# Autodesk Inventor assembly: xy forearm
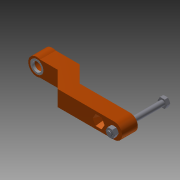
[picture p0: Inventor's stored thumbnail of the model, 180x180]
Saved by Autodesk Inventor 2014 (Build 180170000, 170)
## iProperties
Created: 2013-10-15
Part Number: xy forearm
Document SubType Name: Assembly
Designer: employee
Author: employee
## Documents named in this file (6)
- \\GRISTLE\speco\GitHub\ConceptFORGE\Wally\xy forearm.iam
- \\GRISTLE\speco\GitHub\ConceptFORGE\Wally\xy forearm.ipt
- \\GRISTLE\speco\GitHub\ConceptFORGE\Wally\M3x16.ipt
- \\GRISTLE\speco\GitHub\ConceptFORGE\Wally\6702.ipt
- \\GRISTLE\speco\GitHub\ConceptFORGE\Wally\M8 nut.ipt
- \\GRISTLE\speco\GitHub\ConceptFORGE\Wally\M8x85.ipt
## Components (6 placed, 5 different names)
1. xy forearm:1 — Insert:1, Insert:2, Insert:3, Insert:4, Insert:5
2. Forged Socket Head Cap Screw - Metric M3x0.5 x 16:1 — Insert:1
3. 6702:1 — Insert:2
4. 6702:2 — Insert:3
5. Hex Nut Metric M8 x 1.25:1 — Insert:4
6. M8x85 — Insert:5
## Relationships (5: Insert 5)
- Insert:1 (5 mm): xy forearm:1 ↔ Forged Socket Head Cap Screw - Metric M3x0.5 x 16:1
- Insert:2: xy forearm:1 ↔ 6702:1
- Insert:3: xy forearm:1 ↔ 6702:2
- Insert:4: xy forearm:1 ↔ Hex Nut Metric M8 x 1.25:1
- Insert:5 (51.5 mm): xy forearm:1 ↔ M8x85
